# Autodesk Inventor assembly: Propane Burner Assembly
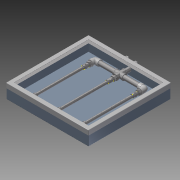
[picture p0: Inventor's stored thumbnail of the model, 180x180]
Saved by Autodesk Inventor 2013 SP2 (Build 170200200, 200)
## iProperties
Created: 2014-05-30
Part Number: Propane Burner Assembly
Document SubType Name: Assembly
Designer: jmw3
Author: jmw3
## Documents named in this file (11)
- F:\NIST\Propane Burner\Propane Burner Assembly.iam
- F:\NIST\Propane Burner\Propane Burner Base.ipt
- F:\NIST\Propane Burner\Propane Burner Lid.ipt
- F:\NIST\Propane Burner\Cross Pipe Fitting ASME B16.3 Class 150.ipt
- F:\NIST\Propane Burner\Welded Pipe Fitting ASTM A312 Schedule 40.ipt
- F:\NIST\Propane Burner\1 in pipe ASTM A 312 - Schedule 40S.ipt
- F:\NIST\Propane Burner\1 in Pipe 90 degree Elbow ASME B16.11 Class 2000.ipt
- F:\NIST\Propane Burner\1 in-.5 in pipe reducer.ipt
- F:\NIST\Propane Burner\.5 in pipe hex coupling.ipt
- F:\NIST\Propane Burner\.5 in pipe.ipt
- F:\NIST\Propane Burner\.5 in pipe cap.ipt
## Components (20 placed, 10 different names)
1. Propane Burner Base:1 — Mate:1, Mate:2, Mate:3, Mate:4, Flush:1, Rotation:1
2. Propane Burner Lid:1 — Mate:1, Mate:2, Mate:3
3. Cross Pipe Fitting ASME B16.3 Class 150:1 — Mate:5, Mate:6, Rotation:2, Mate:7, Mate:8, Rotation:3, Flush:2, Mate:19, Mate:20, Mate:21, Rotation:9, Mate:28, Mate:29, Rotation:10, Rotation:11, Flush:3, Rotation:13
4. Welded Pipe Fitting ASTM A312 Schedule 40:1 — Mate:4, Flush:1, Rotation:1, Mate:5, Mate:6, Rotation:2
5. 1 in pipe ASTM A 312 - Schedule 40S:1 — Mate:7, Mate:8, Rotation:3, Mate:9, Mate:10
6. ASME B16.11 90 Deg Elbow Threaded - Class 2000 1:1 — Mate:9, Flush:2, Mate:10, Mate:11, Mate:12, Rotation:4, Rotation:6, Rotation:7
7. 1 in-.5 in pipe reducer:1 — Mate:11, Mate:12, Rotation:4, Mate:13, Rotation:5, Mate:14
8. .5 in pipe hex coupling:1 — Mate:13, Rotation:5, Rotation:6, Mate:14, Mate:15, Mate:16
9. .5 in pipe:1 — Mate:15, Mate:16, Rotation:7, Mate:17, Mate:18, Rotation:8
10. .5 in pipe cap:1 — Mate:17, Mate:18, Rotation:8
11. 1 in-.5 in pipe reducer:2 — Mate:19, Mate:20, Mate:21, Rotation:9, Mate:22, Mate:23
12. .5 in pipe hex coupling:2 — Mate:34, Mate:35, Mate:36, Mate:37, Rotation:16, Rotation:17
13. .5 in pipe:2 — Mate:24, Mate:25, Rotation:10, Mate:40, Mate:43, Rotation:18
14. 1 in-.5 in pipe reducer:3 — Mate:32, Mate:33, Mate:34, Mate:35, Rotation:15, Rotation:16
15. .5 in pipe hex coupling:3 — Mate:22, Mate:23, Mate:24, Mate:25, Rotation:11
16. .5 in pipe:3 — Mate:36, Mate:37, Rotation:17, Mate:41, Mate:42, Rotation:19
17. 1 in pipe ASTM A 312 - Schedule 40S:2 — Mate:28, Mate:29, Mate:30, Mate:31, Rotation:13, Rotation:14
18. ASME B16.11 90 Deg Elbow Threaded - Class 2000 1:2 — Mate:30, Mate:31, Flush:3, Mate:32, Mate:33, Rotation:14, Rotation:15
19. .5 in pipe cap:4 — Mate:40, Mate:43, Rotation:18
20. .5 in pipe cap:5 — Mate:41, Mate:42, Rotation:19
## Relationships (60: Mate 39, RelateRotation 18, Flush 3)
- Mate:1: Propane Burner Base:1 ↔ Propane Burner Lid:1
- Mate:2: Propane Burner Base:1 ↔ Propane Burner Lid:1
- Mate:3: Propane Burner Base:1 ↔ Propane Burner Lid:1
- Mate:4: Propane Burner Base:1 ↔ Welded Pipe Fitting ASTM A312 Schedule 40:1
- Flush:1 (-25.4 mm): Propane Burner Base:1 ↔ Welded Pipe Fitting ASTM A312 Schedule 40:1
- Rotation:1 [RelateRotation] (1 ul): Propane Burner Base:1 ↔ Welded Pipe Fitting ASTM A312 Schedule 40:1
- Mate:5: Cross Pipe Fitting ASME B16.3 Class 150:1 ↔ Welded Pipe Fitting ASTM A312 Schedule 40:1
- Mate:6: Cross Pipe Fitting ASME B16.3 Class 150:1 ↔ Welded Pipe Fitting ASTM A312 Schedule 40:1
- Rotation:2 [RelateRotation] (1 ul): Cross Pipe Fitting ASME B16.3 Class 150:1 ↔ Welded Pipe Fitting ASTM A312 Schedule 40:1
- Mate:7: Cross Pipe Fitting ASME B16.3 Class 150:1 ↔ 1 in pipe ASTM A 312 - Schedule 40S:1
- Mate:8: Cross Pipe Fitting ASME B16.3 Class 150:1 ↔ 1 in pipe ASTM A 312 - Schedule 40S:1
- Rotation:3 [RelateRotation] (1 ul): Cross Pipe Fitting ASME B16.3 Class 150:1 ↔ 1 in pipe ASTM A 312 - Schedule 40S:1
- Mate:9: 1 in pipe ASTM A 312 - Schedule 40S:1 ↔ ASME B16.11 90 Deg Elbow Threaded - Class 2000 1:1
- Flush:2: Cross Pipe Fitting ASME B16.3 Class 150:1 ↔ ASME B16.11 90 Deg Elbow Threaded - Class 2000 1:1
- Mate:10: 1 in pipe ASTM A 312 - Schedule 40S:1 ↔ ASME B16.11 90 Deg Elbow Threaded - Class 2000 1:1
- Mate:11: ASME B16.11 90 Deg Elbow Threaded - Class 2000 1:1 ↔ 1 in-.5 in pipe reducer:1
- Mate:12: ASME B16.11 90 Deg Elbow Threaded - Class 2000 1:1 ↔ 1 in-.5 in pipe reducer:1
- Rotation:4 [RelateRotation] (1 ul): ASME B16.11 90 Deg Elbow Threaded - Class 2000 1:1 ↔ 1 in-.5 in pipe reducer:1
- Mate:13: 1 in-.5 in pipe reducer:1 ↔ .5 in pipe hex coupling:1
- Rotation:5 [RelateRotation] (1 ul): 1 in-.5 in pipe reducer:1 ↔ .5 in pipe hex coupling:1
- Rotation:6 [RelateRotation] (1 ul): ASME B16.11 90 Deg Elbow Threaded - Class 2000 1:1 ↔ .5 in pipe hex coupling:1
- Mate:14: 1 in-.5 in pipe reducer:1 ↔ .5 in pipe hex coupling:1
- Mate:15: .5 in pipe hex coupling:1 ↔ .5 in pipe:1
- Mate:16: .5 in pipe hex coupling:1 ↔ .5 in pipe:1
- Rotation:7 [RelateRotation] (0.464 ul): ASME B16.11 90 Deg Elbow Threaded - Class 2000 1:1 ↔ .5 in pipe:1
- Mate:17: .5 in pipe:1 ↔ .5 in pipe cap:1
- Mate:18: .5 in pipe:1 ↔ .5 in pipe cap:1
- Rotation:8 [RelateRotation] (1.238 ul): .5 in pipe:1 ↔ .5 in pipe cap:1
- Mate:19: Cross Pipe Fitting ASME B16.3 Class 150:1 ↔ 1 in-.5 in pipe reducer:2
- Mate:20: Cross Pipe Fitting ASME B16.3 Class 150:1 ↔ 1 in-.5 in pipe reducer:2
- Mate:21: Cross Pipe Fitting ASME B16.3 Class 150:1 ↔ 1 in-.5 in pipe reducer:2
- Rotation:9 [RelateRotation] (1 ul): Cross Pipe Fitting ASME B16.3 Class 150:1 ↔ 1 in-.5 in pipe reducer:2
- Mate:22: 1 in-.5 in pipe reducer:2 ↔ .5 in pipe hex coupling:3
- Mate:23: 1 in-.5 in pipe reducer:2 ↔ .5 in pipe hex coupling:3
- Mate:24: .5 in pipe:2 ↔ .5 in pipe hex coupling:3
- Mate:25: .5 in pipe:2 ↔ .5 in pipe hex coupling:3
- Mate:28: Cross Pipe Fitting ASME B16.3 Class 150:1 ↔ 1 in pipe ASTM A 312 - Schedule 40S:2
- Mate:29: Cross Pipe Fitting ASME B16.3 Class 150:1 ↔ 1 in pipe ASTM A 312 - Schedule 40S:2
- Rotation:10 [RelateRotation] (0.475 ul): Cross Pipe Fitting ASME B16.3 Class 150:1 ↔ .5 in pipe:2
- Rotation:11 [RelateRotation] (0.638 ul): Cross Pipe Fitting ASME B16.3 Class 150:1 ↔ .5 in pipe hex coupling:3
- Mate:30: 1 in pipe ASTM A 312 - Schedule 40S:2 ↔ ASME B16.11 90 Deg Elbow Threaded - Class 2000 1:2
- Mate:31: 1 in pipe ASTM A 312 - Schedule 40S:2 ↔ ASME B16.11 90 Deg Elbow Threaded - Class 2000 1:2
- Flush:3: Cross Pipe Fitting ASME B16.3 Class 150:1 ↔ ASME B16.11 90 Deg Elbow Threaded - Class 2000 1:2
- Mate:32: 1 in-.5 in pipe reducer:3 ↔ ASME B16.11 90 Deg Elbow Threaded - Class 2000 1:2
- Mate:33: 1 in-.5 in pipe reducer:3 ↔ ASME B16.11 90 Deg Elbow Threaded - Class 2000 1:2
- Mate:34: .5 in pipe hex coupling:2 ↔ 1 in-.5 in pipe reducer:3
- Mate:35: .5 in pipe hex coupling:2 ↔ 1 in-.5 in pipe reducer:3
- Mate:36: .5 in pipe hex coupling:2 ↔ .5 in pipe:3
- Mate:37: .5 in pipe hex coupling:2 ↔ .5 in pipe:3
- Rotation:13 [RelateRotation] (0.743 ul): Cross Pipe Fitting ASME B16.3 Class 150:1 ↔ 1 in pipe ASTM A 312 - Schedule 40S:2
- Rotation:14 [RelateRotation] (1.376 ul): 1 in pipe ASTM A 312 - Schedule 40S:2 ↔ ASME B16.11 90 Deg Elbow Threaded - Class 2000 1:2
- Rotation:15 [RelateRotation] (0.276 ul): 1 in-.5 in pipe reducer:3 ↔ ASME B16.11 90 Deg Elbow Threaded - Class 2000 1:2
- Rotation:16 [RelateRotation] (1 ul): .5 in pipe hex coupling:2 ↔ 1 in-.5 in pipe reducer:3
- Rotation:17 [RelateRotation] (0.743 ul): .5 in pipe hex coupling:2 ↔ .5 in pipe:3
- Mate:40: .5 in pipe:2 ↔ .5 in pipe cap:4
- Mate:41: .5 in pipe:3 ↔ .5 in pipe cap:5
- Mate:42: .5 in pipe:3 ↔ .5 in pipe cap:5
- Mate:43: .5 in pipe:2 ↔ .5 in pipe cap:4
- Rotation:18 [RelateRotation] (1.238 ul): .5 in pipe:2 ↔ .5 in pipe cap:4
- Rotation:19 [RelateRotation] (1.452 ul): .5 in pipe:3 ↔ .5 in pipe cap:5
